# Autodesk Inventor assembly: E2Assembly
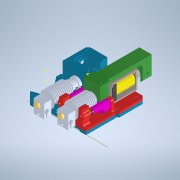
[picture p0: Inventor's stored thumbnail of the model, 180x180]
Saved by Autodesk Inventor 2020 (Build 240168000, 168)
## iProperties
Created: 2019-11-05
Part Number: E2Assembly
Document SubType Name: Assembly
Designer: Owner
Author: Owner
## Documents named in this file (9)
- C:\Users\Owner\Documents\PepCo\05 Nov 2019 - MK3PRO P1 - ParkerExportL\MK3PRO P1\E2\E2Assembly.iam
- C:\Users\Owner\Documents\PepCo\05 Nov 2019 - MK3PRO P1 - ParkerExportL\MK3PRO P1\E2\BackPlate.ipt
- C:\Users\Owner\Documents\PepCo\Extruder\Solenoid Assembly.iam
- C:\Users\Owner\Documents\PepCo\05 Nov 2019 - MK3PRO P1 - ParkerExportL\MK3PRO P1\E-Axis\Extruder Back V1.2.ipt
- C:\Users\Owner\Documents\PepCo\05 Nov 2019 - MK3PRO P1 - ParkerExportL\MK3PRO P1\E-Axis\E3D_V6.ipt
- C:\Users\Owner\Documents\PepCo\30 Oct 2019 - MK3PRO P1 - ParkerExportL\MK3PRO P1\Part7.ipt
- C:\Users\Owner\Documents\PepCo\30 Oct 2019 - MK3PRO P1 - ParkerExportL\MK3PRO P1\part6.ipt
- C:\Users\Owner\Documents\PepCo\05 Nov 2019 - MK3PRO P1 - ParkerExportL\MK3PRO P1\E2\91595A185_METRIC ALLOY STEEL DOWEL PIN.ipt
- C:\Users\Owner\Documents\PepCo\05 Nov 2019 - MK3PRO P1 - ParkerExportL\MK3PRO P1\E2\Bushing.ipt
## Components (11 placed, 8 different names)
1. BackPlate:1 — Mate:2, Mate:3, Mate:4, Flush:1, Flush:2, Angle:4, Insert:1, Insert:2, Mate:13
2. Solenoid Assembly:1 [sub-assembly] — Mate:2, Mate:3, Mate:7, Mate:8, Mate:13
3. Extruder Back V1.2:1 — Mate:4, Flush:1, Flush:2, Mate:5, Mate:6
4. E3D_V6:1 — Mate:5, Mate:6, Angle:3
5. E3D_V6:2 — Mate:9, Mate:10, Angle:2, Angle:3, Angle:4
6. Part7:1 — Mate:9, Mate:10, Mate:11, Mate:12, Angle:1, Mate:14, Mate:15, Mate:16, Mate:17
7. part6:1 — Mate:7, Mate:8, Mate:11, Mate:12, Angle:1, Angle:2
8. 91595A185_METRIC ALLOY STEEL DOWEL PIN:1 — Insert:1
9. 91595A185_METRIC ALLOY STEEL DOWEL PIN:2 — Insert:2
10. Bushing:1 — Mate:16, Mate:17
11. Bushing:2 — Mate:14, Mate:15
## Relationships (24: Mate 16, Angle 4, Flush 2, Insert 2)
- Mate:2: BackPlate:1 ↔ Solenoid Assembly:1
- Mate:3: BackPlate:1 ↔ Solenoid Assembly:1
- Mate:4: BackPlate:1 ↔ Extruder Back V1.2:1
- Flush:1: BackPlate:1 ↔ Extruder Back V1.2:1
- Flush:2: BackPlate:1 ↔ Extruder Back V1.2:1
- Mate:5: Extruder Back V1.2:1 ↔ E3D_V6:1
- Mate:6: Extruder Back V1.2:1 ↔ E3D_V6:1
- Mate:7: Solenoid Assembly:1 ↔ part6:1
- Mate:8: Solenoid Assembly:1 ↔ part6:1
- Mate:9: E3D_V6:2 ↔ Part7:1
- Mate:10: E3D_V6:2 ↔ Part7:1
- Mate:11: Part7:1 ↔ part6:1
- Mate:12: Part7:1 ↔ part6:1
- Angle:1 (180 deg): Part7:1 ↔ part6:1
- Angle:2 (0 deg): E3D_V6:2 ↔ part6:1
- Angle:3 (0 deg): E3D_V6:1 ↔ E3D_V6:2
- Angle:4 (0 deg): BackPlate:1 ↔ E3D_V6:2
- Insert:1 (-1 mm): BackPlate:1 ↔ 91595A185_METRIC ALLOY STEEL DOWEL PIN:1
- Insert:2 (1 mm): BackPlate:1 ↔ 91595A185_METRIC ALLOY STEEL DOWEL PIN:2
- Mate:13: BackPlate:1 ↔ Solenoid Assembly:1
- Mate:14: Part7:1 ↔ Bushing:2
- Mate:15: Part7:1 ↔ Bushing:2
- Mate:16: Part7:1 ↔ Bushing:1
- Mate:17: Part7:1 ↔ Bushing:1
